# Autodesk Inventor assembly: NASA-20-MM
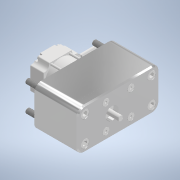
[picture p0: Inventor's stored thumbnail of the model, 180x180]
Saved by Autodesk Inventor 2020 (Build 240168000, 168)
## iProperties
Created: 2019-09-22
Part Number: NASA-20-MM
Document SubType Name: Assembly
Designer: Rick Szalay
Description: MOTOR MOUNT
Author: Rick Szalay
## Documents named in this file (6)
- C:\Users\Vitaliy\Documents\Robotics\NASA-20\NASA-20\MM\NASA-20-MM.iam
- C:\Users\Vitaliy\Documents\Robotics\NASA-20\NASA-20\MM\NASA-20-MM-MB-01.ipt
- C:\Users\Vitaliy\Documents\Robotics\NASA-20\NASA-20\A428.ipt
- C:\Users\Vitaliy\Documents\Robotics\NASA-20\NASA-20\MM\NASA-20-MM-MP-01.ipt
- C:\Users\Vitaliy\Documents\Robotics\NASA-20\NASA-20\MM\MM-MMount_to_Frame-Bolt.ipt
- C:\Users\Vitaliy\Documents\Robotics\NASA-20\NASA-20\MM\MM-MMount_to_Motor-CS_Bolt-.ipt
## Components (11 placed, 5 different names)
1. NASA-20-MM-MB-01:1 — Flush:1, Mate:1, Mate:2, Mate:3, Flush:2, Flush:3
2. A428:1 — Flush:1, Mate:1, Mate:2
3. NASA-20-MM-MP-01:1 — Mate:3, Flush:2, Flush:3, Mate:4, Mate:5, Mate:6, Mate:7, Mate:8, Mate:9, Mate:10, Mate:11, Mate:12, Mate:13, Mate:14, Mate:15, Flush:4, Flush:5, Flush:6, Flush:7
4. MM-MMount_to_Frame-Bolt:1 — Mate:4, Mate:8
5. MM-MMount_to_Frame-Bolt:2 — Mate:5, Mate:9
6. MM-MMount_to_Frame-Bolt:3 — Mate:6, Mate:11
7. MM-MMount_to_Frame-Bolt:4 — Mate:7, Mate:10
8. MM-MMount_to_Motor-CS_Bolt-:1 — Mate:13, Flush:7
9. MM-MMount_to_Motor-CS_Bolt-:2 — Mate:14, Flush:4
10. MM-MMount_to_Motor-CS_Bolt-:3 — Mate:15, Flush:6
11. MM-MMount_to_Motor-CS_Bolt-:4 — Mate:12, Flush:5
## Relationships (22: Mate 15, Flush 7)
- Flush:1: NASA-20-MM-MB-01:1 ↔ A428:1
- Mate:1: NASA-20-MM-MB-01:1 ↔ A428:1
- Mate:2: NASA-20-MM-MB-01:1 ↔ A428:1
- Mate:3: NASA-20-MM-MB-01:1 ↔ NASA-20-MM-MP-01:1
- Flush:2: NASA-20-MM-MB-01:1 ↔ NASA-20-MM-MP-01:1
- Flush:3: NASA-20-MM-MB-01:1 ↔ NASA-20-MM-MP-01:1
- Mate:4: NASA-20-MM-MP-01:1 ↔ MM-MMount_to_Frame-Bolt:1
- Mate:5: NASA-20-MM-MP-01:1 ↔ MM-MMount_to_Frame-Bolt:2
- Mate:6: NASA-20-MM-MP-01:1 ↔ MM-MMount_to_Frame-Bolt:3
- Mate:7: NASA-20-MM-MP-01:1 ↔ MM-MMount_to_Frame-Bolt:4
- Mate:8: NASA-20-MM-MP-01:1 ↔ MM-MMount_to_Frame-Bolt:1
- Mate:9: NASA-20-MM-MP-01:1 ↔ MM-MMount_to_Frame-Bolt:2
- Mate:10: NASA-20-MM-MP-01:1 ↔ MM-MMount_to_Frame-Bolt:4
- Mate:11: NASA-20-MM-MP-01:1 ↔ MM-MMount_to_Frame-Bolt:3
- Mate:12: NASA-20-MM-MP-01:1 ↔ MM-MMount_to_Motor-CS_Bolt-:4
- Mate:13: NASA-20-MM-MP-01:1 ↔ MM-MMount_to_Motor-CS_Bolt-:1
- Mate:14: NASA-20-MM-MP-01:1 ↔ MM-MMount_to_Motor-CS_Bolt-:2
- Mate:15: NASA-20-MM-MP-01:1 ↔ MM-MMount_to_Motor-CS_Bolt-:3
- Flush:4: NASA-20-MM-MP-01:1 ↔ MM-MMount_to_Motor-CS_Bolt-:2
- Flush:5: NASA-20-MM-MP-01:1 ↔ MM-MMount_to_Motor-CS_Bolt-:4
- Flush:6: NASA-20-MM-MP-01:1 ↔ MM-MMount_to_Motor-CS_Bolt-:3
- Flush:7: NASA-20-MM-MP-01:1 ↔ MM-MMount_to_Motor-CS_Bolt-:1
